# Autodesk Inventor assembly: Робот
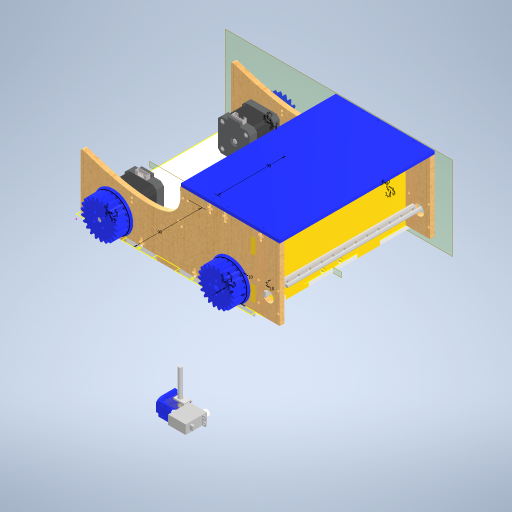
[picture p0: Inventor's stored thumbnail of the model, 512x512]
Saved by Autodesk Inventor 2024.2 (Build 282272000, 272)
## iProperties
Created: 2026-01-27
Part Number: Робот
Document SubType Name: Assembly
Designer: Service
d4: 0,000 мм
Author: Service
## Documents named in this file (11)
- C:\Users\Service\Documents\Artist-v2\3D\Робот.iam
- C:\Users\Service\Documents\Artist-v2\3D\Низ робота.ipt
- C:\Users\Service\Documents\Artist-v2\3D\бок.ipt
- C:\Users\Service\Documents\Artist-v2\3D\перед.ipt
- C:\Users\Service\Documents\Artist-v2\3D\NEMA17 42-40.ipt
- C:\Users\Service\Documents\Artist-v2\3D\Шестерня.ipt
- C:\Users\Service\Documents\Artist-v2\3D\stl\крепеж валика.ipt
- C:\Users\Service\Documents\Artist-v2\3D\dxf\спиралька.ipt
- C:\Users\Service\Documents\Artist-v2\3D\MGN7.ipt
- C:\Users\Service\Documents\Artist-v2\3D\stl\крышка.ipt
- C:\Users\Service\Documents\Artist-v2\3D\каретка.iam
## Components (15 placed, 10 different names)
1. Низ робота:1 — Совмещение:2, Заподлицо:3, Совмещение:12, Заподлицо:9, Заподлицо:23, Заподлицо:25, Совмещение:47, Заподлицо:26, Заподлицо:27
2. бок:1 — Совмещение:4, Совмещение:5, Совмещение:13, Совмещение:42, Совмещение:43, Совмещение:47, Заподлицо:26, Заподлицо:27, Заподлицо:28
3. бок:2 — Совмещение:2, Заподлицо:3, Совмещение:6, Совмещение:7, Совмещение:8, Совмещение:10, Совмещение:19, Совмещение:20, Заподлицо:21, Заподлицо:22, Совмещение:45, Заподлицо:24, Совмещение:48, Заподлицо:29
4. перед:1 — Заподлицо:23, Заподлицо:24, Заподлицо:25
5. NEMA17 42-40:1 — Совмещение:4, Совмещение:5, Совмещение:12, Совмещение:14
6. NEMA17 42-40:2 — Совмещение:6, Совмещение:7, Совмещение:8, Совмещение:9
7. Шестерня:1 — Совмещение:13, Совмещение:14
8. Шестерня:2 — Совмещение:42, Совмещение:43
9. Шестерня:3 — Совмещение:19, Совмещение:20
10. Шестерня:4 — Совмещение:9, Совмещение:10
11. крепеж валика:1 — Заподлицо:9
12. спиралька:1 — Заподлицо:21, Заподлицо:22
13. MGN7:1 — Совмещение:45
14. крышка:1 — Совмещение:48, Заподлицо:28, Заподлицо:29
15. каретка:1 [sub-assembly]
## Relationships (29: Mate 18, Flush 11)
- Совмещение:2 [Mate]: Низ робота:1 ↔ бок:2
- Заподлицо:3 [Flush]: Низ робота:1 ↔ бок:2
- Совмещение:4 [Mate]: бок:1 ↔ NEMA17 42-40:1
- Совмещение:5 [Mate]: бок:1 ↔ NEMA17 42-40:1
- Совмещение:6 [Mate]: бок:2 ↔ NEMA17 42-40:2
- Совмещение:7 [Mate]: бок:2 ↔ NEMA17 42-40:2
- Совмещение:8 [Mate]: бок:2 ↔ NEMA17 42-40:2
- Совмещение:9 [Mate]: NEMA17 42-40:2 ↔ Шестерня:4
- Совмещение:10 [Mate]: бок:2 ↔ Шестерня:4
- Совмещение:12 [Mate]: Низ робота:1 ↔ NEMA17 42-40:1
- Совмещение:13 [Mate]: бок:1 ↔ Шестерня:1
- Совмещение:14 [Mate]: NEMA17 42-40:1 ↔ Шестерня:1
- Совмещение:19 [Mate]: бок:2 ↔ Шестерня:3
- Совмещение:20 [Mate]: бок:2 ↔ Шестерня:3
- Заподлицо:9 [Flush]: Низ робота:1 ↔ крепеж валика:1
- Совмещение:42 [Mate]: бок:1 ↔ Шестерня:2
- Совмещение:43 [Mate]: бок:1 ↔ Шестерня:2
- Заподлицо:21 [Flush]: бок:2 ↔ спиралька:1
- Заподлицо:22 [Flush]: бок:2 ↔ спиралька:1
- Совмещение:45 [Mate]: бок:2 ↔ MGN7:1
- Заподлицо:23 [Flush]: Низ робота:1 ↔ перед:1
- Заподлицо:24 [Flush]: бок:2 ↔ перед:1
- Заподлицо:25 [Flush]: Низ робота:1 ↔ перед:1
- Совмещение:47 [Mate]: Низ робота:1 ↔ бок:1
- Заподлицо:26 [Flush]: Низ робота:1 ↔ бок:1
- Заподлицо:27 [Flush]: Низ робота:1 ↔ бок:1
- Совмещение:48 [Mate]: бок:2 ↔ крышка:1
- Заподлицо:28 [Flush]: бок:1 ↔ крышка:1
- Заподлицо:29 [Flush]: бок:2 ↔ крышка:1
